# Autodesk Inventor assembly: SCSTR10-10
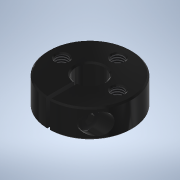
[picture p0: Inventor's stored thumbnail of the model, 180x180]
Saved by Autodesk Inventor 2022.3 (Build 263350000, 350)
## iProperties
Category: PARTsolutions
Company: MISUMI
Created: 2019-10-22
Part Number: SCSTR10-10
Catalog Web Link: www.cadenas.de
Description: SCST, PSCST, SSCST, SCSTR, PSCSTR, SSCSTR-Shaft Collars - 3 Holes/3 Taps
Vendor: MISUMI
Document SubType Name: Assembly
Designer: psadmin
Manufacturer: MISUMI
PSOL_IDENT_0: {$CADENAS_DATA\23d-libs\misumi\metric\03_set_collars\scst_asmtab.prj},223 {VTYP=3D},{STYP=ASSTAB},{N
PSOL_IDENT_1: B=SCSTR10-10},{LINA=SCSTR10-10},{NN=SCST, PSCST, SSCST, SCSTR, PSCSTR, SSCSTR},{DATE=04.10.2019 12:5
PSOL_IDENT_2: 4:03},{GEOMDATE=30.10.2015 01:45:58},{VERSION=},{LINEID=60},{WBVAR=TS,MAT,ST,BS},{WBNUMERIC=BS}  {NB=
PSOL_IDENT_3: SCSTR10-10},{LINA=SCSTR10-10},{KT=DUMMY},{PN=SCSTR10-10},{TYPE=SCSTR},{TS=3T},{TSALG= '3H' , '3-Hole'
PSOL_IDENT_4: , '3T' , '3-Tapped' },{MAT=S45C},{ST=BO},{STALG= 'BO' , 'Black Oxide' , 'ENP' , 'Electroless Nickel
PSOL_IDENT_5: Plating' },{AC=Hex Socket Head Cap Screw 1 pc.},{ACMAT=4137 Alloy Steel},{D=10},{BS=10},{BALG= 8 ,
PSOL_IDENT_6: 10 },{D1=30},{M=M4},{M3D=4},{DD=4.5},{R=3.75},{W=1.5},{X=9.0},{Y=5},{P=20},{C=0.5},{S=0.0},{M1=M5},{
PSOL_IDENT_7: M13D=5},{L=15},{PPATH=scst/scst_templ.prj}
NN: SCST, PSCST, SSCST, SCSTR, PSCSTR, SSCSTR
NT: Shaft Collars - 3 Holes/3 Taps
NB: SCSTR10-10
NBSYN: $PN.
LINA: SCSTR10-10
PN: SCSTR10-10
TS: 3-Tapped
MAT: 1045 Carbon Steel
ST: Black Oxide
AC: Hex Socket Head Cap Screw 1 pc.
ACMAT: 4137 Alloy Steel
D: 10
BS: 10
D1: 30
M: M4
DD: 4.5
R: 3.75
W: 1.5
X: 9
Y: 5
P: 20
C: 0.5
S: 0
M1: M5
SUPPLIER: MISUMI
ARTICLENO: SCSTR10-10
BOMINFO: SCSTR10-10
CREATOR: CADENAS GmbH
Title: SCSTR10-10
Author: Cadenas PARTsolutions
Comments: Shaft Collars - 3 Holes/3 Taps
## Documents named in this file (3)
- C:\Users\YusukeKunita\Documents\GrabCAD\Development\BasicParts\SetCollar\SCSTR10-10\SCSTR10-10.iam
- C:\Users\YusukeKunita\Documents\GrabCAD\Development\BasicParts\SetCollar\SCSTR10-10\SCSTR10-10b.ipt
- C:\Users\YusukeKunita\Documents\GrabCAD\Development\BasicParts\SetCollar\SCSTR10-10\BOLT4-15.ipt
## Components (2 placed, 2 different names)
1. SCSTR10-10b:1 — to_bolt_XY@1 <-> to_cp_XY@2, to_bolt_Z@1 <-> to_cp_Z@2, to_bolt_YZ@1 <-> to_cp_YZ@2
2. BOLT4-15:1 — to_bolt_XY@1 <-> to_cp_XY@2, to_bolt_Z@1 <-> to_cp_Z@2, to_bolt_YZ@1 <-> to_cp_YZ@2
## Relationships (3: Mate 2, Angle 1)
- to_bolt_XY@1 <-> to_cp_XY@2 [Mate]: SCSTR10-10b:1 ↔ BOLT4-15:1
- to_bolt_Z@1 <-> to_cp_Z@2 [Mate]: SCSTR10-10b:1 ↔ BOLT4-15:1
- to_bolt_YZ@1 <-> to_cp_YZ@2 [Angle] (0 deg): SCSTR10-10b:1 ↔ BOLT4-15:1
